# Autodesk Inventor assembly: IceKeysV1
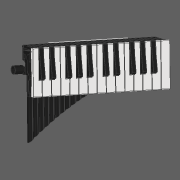
[picture p0: Inventor's stored thumbnail of the model, 180x180]
Saved by Autodesk Inventor 2020 (Build 240168000, 168)
## iProperties
Created: 2019-12-01
Part Number: IceKeysV1
Document SubType Name: Assembly
Designer: Isaac Newcomb
Mass: 549.637 g
Surface Area: 4250.67 cm^2
Volume: 535.657 cm^3
Density: 1.0261 g/cm^3
Project: Ice Keys
Author: Isaac Newcomb
## Documents named in this file (18)
- Z:\Ice Keys\V1\IceKeysV1.iam
- Z:\Ice Keys\V1\Manifold0_Lower.ipt
- Z:\Ice Keys\V1\BlackKey0.ipt
- Z:\Ice Keys\V1\Lever1.ipt
- Z:\Ice Keys\V1\DKey0.ipt
- Z:\Ice Keys\V1\PostValve1_Upper.ipt
- Z:\Ice Keys\V1\PostValve1_Lower.ipt
- Z:\Ice Keys\V1\Manifold0_Upper.ipt
- Z:\Ice Keys\V1\HandPlate0.ipt
- Z:\Ice Keys\V1\PostValve1.ipt
- Z:\Ice Keys\V1\CKey0.ipt
- Z:\Ice Keys\V1\EKey0.ipt
- Z:\Ice Keys\V1\FKey0.ipt
- Z:\Ice Keys\V1\GKey0.ipt
- Z:\Ice Keys\V1\AKey0.ipt
- Z:\Ice Keys\V1\BKey0.ipt
- Z:\Ice Keys\V1\CKey0_Top.ipt
- Z:\Ice Keys\V1\TuningPlug0.ipt
## Components (56 placed, 16 different names)
1. Manifold0_Lower:1 — Rigid:5, Mate:7, Mate:8, Rigid:6
2. PostValve1_Lower:1 — Rigid:4, Rotational:1, Rotational:2, Rigid:5, Mate:4, Mate:5, Mate:6, Flush:1, Rotational:3, Rotational:4, Rotational:5, Rotational:6, Rotational:7, Rotational:9
3. PostValve1_Upper:1 — Rigid:4, Rotational:10, Rotational:8, Cylindrical:2
4. Manifold0_Upper:1 — Rigid:6
5. HandPlate0:1 — Mate:7, Mate:8, Flush:1
6. CKey0_Top:13 — Rotational:8
7. TuningPlug0:1 — Cylindrical:2
8. CKey0:1 — Rotational:3, Rigid:7
9. DKey0:1 — Rotational:2
10. EKey0:2 — Rotational:4
11. FKey0:3 — Rotational:5
12. GKey0:4 — Rotational:6
13. AKey0:5 — Rotational:7
14. BKey0:6 — Rotational:10
15. CKey0:7
16. DKey0:2
17. EKey0:8
18. FKey0:9
19. GKey0:10
20. AKey0:11
21. BKey0:12
22. Lever1:1 — Rigid:7
23. Lever1:2
24. Lever1:3
25. Lever1:4
26. Lever1:5
27. Lever1:6
28. Lever1:7
29. Lever1:8
30. Lever1:9
31. Lever1:10
32. Lever1:11
33. Lever1:12
34. Lever1:13
35. Lever1:14
36. Lever1:15
37. Lever1:16
38. Lever1:17
39. Lever1:18
40. Lever1:19
41. Lever1:20
42. Lever1:21
43. Lever1:22
44. Lever1:23
45. Lever1:24
46. Lever1:25
47. BlackKey0:1 — Rotational:1
48. BlackKey0:2
49. BlackKey0:3 — Rotational:9
50. BlackKey0:4
51. BlackKey0:5
52. BlackKey0:6
53. BlackKey0:7
54. BlackKey0:8
55. BlackKey0:9
56. BlackKey0:10
## Component patterns: White Keys (2 elements), Key Backs (25 elements), Black Keys (2 elements), (2 elements, first: BlackKey0:1), (3 elements, first: BlackKey0:3), Component Pattern 3:2 (2 elements), Component Pattern 4:2 (3 elements)
## Relationships (21: RevoluteJoint 10, Mate 5, WeldJoint 4, Flush 1, CylindricalJoint 1)
- Rigid:4 [WeldJoint]: PostValve1_Lower:1 ↔ PostValve1_Upper:1
- Rotational:1 [RevoluteJoint]: PostValve1_Lower:1 ↔ BlackKey0:1
- Rotational:2 [RevoluteJoint]: PostValve1_Lower:1 ↔ DKey0:1
- Rigid:5 [WeldJoint]: Manifold0_Lower:1 ↔ PostValve1_Lower:1
- Mate:4: PostValve1_Lower:1
- Mate:5: PostValve1_Lower:1
- Mate:6: PostValve1_Lower:1
- Mate:7: Manifold0_Lower:1 ↔ HandPlate0:1
- Mate:8: Manifold0_Lower:1 ↔ HandPlate0:1
- Flush:1 (60.375 mm): PostValve1_Lower:1 ↔ HandPlate0:1
- Rigid:6 [WeldJoint]: Manifold0_Lower:1 ↔ Manifold0_Upper:1
- Rotational:3 [RevoluteJoint]: PostValve1_Lower:1 ↔ CKey0:1
- Rotational:4 [RevoluteJoint]: PostValve1_Lower:1 ↔ EKey0:2
- Rotational:5 [RevoluteJoint]: PostValve1_Lower:1 ↔ FKey0:3
- Rotational:6 [RevoluteJoint]: PostValve1_Lower:1 ↔ GKey0:4
- Rotational:7 [RevoluteJoint]: PostValve1_Lower:1 ↔ AKey0:5
- Rotational:10 [RevoluteJoint]: PostValve1_Upper:1 ↔ BKey0:6
- Rotational:8 [RevoluteJoint]: PostValve1_Upper:1 ↔ CKey0_Top:13
- Rigid:7 [WeldJoint] (0.1 mm): CKey0:1 ↔ Lever1:1
- Rotational:9 [RevoluteJoint]: PostValve1_Lower:1 ↔ BlackKey0:3
- Cylindrical:2: PostValve1_Upper:1 ↔ TuningPlug0:1
## Named parameters: chanWidth = 12 mm, keyCount = 25, resoWallThick = 0.75 mm
